# Autodesk Inventor assembly: POM_T5_15
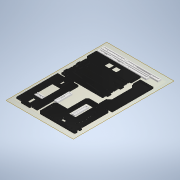
[picture p0: Inventor's stored thumbnail of the model, 180x180]
Saved by Autodesk Inventor 2020 (Build 240168000, 168)
## iProperties
Created: 2021-08-27
Part Number: POM_T5_15
Document SubType Name: Assembly
Designer: Masato
Author: Masato
## Documents named in this file (16)
- C:\Inventor\SUSTAINA-OP_0521\Cam\POM_T5_15.iam
- C:\Inventor\SUSTAINA-OP_0521\Cam\DisposableBoard.ipt
- C:\Inventor\SUSTAINA-OP_0521\UpperBody\Cockpit\Cockpit_battery_bottom_frame.ipt
- C:\Inventor\SUSTAINA-OP_0521\UpperBody\Cockpit\Cockpit_battery_front_frame.ipt
- C:\Inventor\SUSTAINA-OP_0521\UpperBody\Cockpit\Cockpit_side_frame.ipt
- C:\Inventor\SUSTAINA-OP_0521\UpperBody\Cockpit\Cockpit_back_frame.ipt
- C:\Inventor\SUSTAINA-OP_0521\UpperBody\Cockpit\Cockpit_battery_back_door.ipt
- C:\Inventor\SUSTAINA-OP_0521\UpperBody\Cockpit\Cockpit_top_frame.ipt
- C:\Inventor\SUSTAINA-OP_0521\Jig\Cockpit_side_frame_Jig.ipt
- C:\Inventor\SUSTAINA-OP_0521\Jig\Cockpit_battery_bottom_frame_Jig.ipt
- C:\Inventor\SUSTAINA-OP_0521\Jig\Cockpit_battery_back_door_Jig.ipt
- C:\Inventor\SUSTAINA-OP_0521\Jig\Cockpit_battery_front_frame_Jig.ipt
- C:\Inventor\SUSTAINA-OP_0521\Jig\Cockpit_battery_front_frame_Jig_2.ipt
- C:\Inventor\SUSTAINA-OP_0521\Jig\Cockpit_front_frame_Jig.ipt
- C:\Inventor\SUSTAINA-OP_0521\Jig\Cockpit_back_frame_Jig.ipt
- C:\Inventor\SUSTAINA-OP_0520\Jig\Cockpit_carrier_board_frame_Jig.ipt
## Components (15 placed, 15 different names)
1. DisposableBoard:1 — メイト:2, メイト:1, フラッシュ:1, フラッシュ:2, メイト:4, メイト:5, メイト:6, フラッシュ:3, フラッシュ:4, フラッシュ:6, メイト:7, メイト:8, メイト:12, メイト:14, メイト:17, メイト:20, メイト:26, メイト:27, メイト:28, メイト:32, メイト:33
2. Cockpit_side_frame:1 — メイト:5, フラッシュ:5, フラッシュ:6, フラッシュ:7, メイト:11, メイト:18, メイト:24, メイト:25
3. Cockpit_back_frame:1 — メイト:4, フラッシュ:3, フラッシュ:4, フラッシュ:5, フラッシュ:8, メイト:9, メイト:15, メイト:16, メイト:19
4. Cockpit_battery_back_door:1 — メイト:6, フラッシュ:7, メイト:11
5. Cockpit_battery_bottom_frame:1 — メイト:7, フラッシュ:8, フラッシュ:9, メイト:10, フラッシュ:10, メイト:13
6. Cockpit_battery_front_frame:1 — メイト:8, フラッシュ:9, メイト:9, メイト:10
7. Cockpit_top_frame:2 — メイト:12, フラッシュ:10, メイト:13, フラッシュ:13, メイト:29
8. Cockpit_side_frame_Jig:1 — メイト:14, メイト:15, メイト:16
9. Cockpit_battery_bottom_frame_Jig:1 — メイト:17, メイト:18, メイト:19
10. Cockpit_battery_back_door_Jig:1 — メイト:20, メイト:24, メイト:25
11. Cockpit_battery_front_frame_Jig:1 — メイト:26, フラッシュ:13, メイト:29, メイト:30, フラッシュ:14, フラッシュ:16, メイト:34
12. Cockpit_battery_front_frame_Jig_2:1 — メイト:27, メイト:30, フラッシュ:14, フラッシュ:15, メイト:31
13. Cockpit_front_frame_Jig:1 — メイト:28, フラッシュ:15, メイト:31
14. Cockpit_back_frame_Jig:1 — メイト:32, フラッシュ:16, メイト:34, フラッシュ:17, メイト:35
15. Cockpit_carrier_board_frame_Jig:1 — メイト:33, フラッシュ:17, メイト:35
## Relationships (46: Mate 31, Flush 15)
- メイト:2 [Mate]: DisposableBoard:1
- メイト:1 [Mate]: DisposableBoard:1
- フラッシュ:1 [Flush]: DisposableBoard:1
- フラッシュ:2 [Flush]: DisposableBoard:1
- メイト:4 [Mate]: DisposableBoard:1 ↔ Cockpit_back_frame:1
- メイト:5 [Mate]: DisposableBoard:1 ↔ Cockpit_side_frame:1
- メイト:6 [Mate]: DisposableBoard:1 ↔ Cockpit_battery_back_door:1
- フラッシュ:3 [Flush] (2 mm): DisposableBoard:1 ↔ Cockpit_back_frame:1
- フラッシュ:4 [Flush] (2 mm): DisposableBoard:1 ↔ Cockpit_back_frame:1
- フラッシュ:5 [Flush]: Cockpit_side_frame:1 ↔ Cockpit_back_frame:1
- フラッシュ:6 [Flush] (2 mm): DisposableBoard:1 ↔ Cockpit_side_frame:1
- フラッシュ:7 [Flush]: Cockpit_side_frame:1 ↔ Cockpit_battery_back_door:1
- メイト:7 [Mate]: DisposableBoard:1 ↔ Cockpit_battery_bottom_frame:1
- メイト:8 [Mate]: DisposableBoard:1 ↔ Cockpit_battery_front_frame:1
- フラッシュ:8 [Flush]: Cockpit_back_frame:1 ↔ Cockpit_battery_bottom_frame:1
- フラッシュ:9 [Flush]: Cockpit_battery_bottom_frame:1 ↔ Cockpit_battery_front_frame:1
- メイト:9 [Mate] (2.5 mm): Cockpit_back_frame:1 ↔ Cockpit_battery_front_frame:1
- メイト:10 [Mate] (2.5 mm): Cockpit_battery_bottom_frame:1 ↔ Cockpit_battery_front_frame:1
- メイト:11 [Mate] (2.5 mm): Cockpit_side_frame:1 ↔ Cockpit_battery_back_door:1
- メイト:12 [Mate]: DisposableBoard:1 ↔ Cockpit_top_frame:2
- フラッシュ:10 [Flush]: Cockpit_battery_bottom_frame:1 ↔ Cockpit_top_frame:2
- メイト:13 [Mate] (2.5 mm): Cockpit_battery_bottom_frame:1 ↔ Cockpit_top_frame:2
- メイト:14 [Mate]: DisposableBoard:1 ↔ Cockpit_side_frame_Jig:1
- メイト:15 [Mate] (2.5 mm): Cockpit_back_frame:1 ↔ Cockpit_side_frame_Jig:1
- メイト:16 [Mate] (3.5 mm): Cockpit_back_frame:1 ↔ Cockpit_side_frame_Jig:1
- メイト:17 [Mate]: DisposableBoard:1 ↔ Cockpit_battery_bottom_frame_Jig:1
- メイト:18 [Mate] (2.5 mm): Cockpit_side_frame:1 ↔ Cockpit_battery_bottom_frame_Jig:1
- メイト:19 [Mate] (2.5 mm): Cockpit_back_frame:1 ↔ Cockpit_battery_bottom_frame_Jig:1
- メイト:20 [Mate]: DisposableBoard:1 ↔ Cockpit_battery_back_door_Jig:1
- メイト:24 [Mate] (4.5 mm): Cockpit_side_frame:1 ↔ Cockpit_battery_back_door_Jig:1
- メイト:25 [Mate] (7 mm): Cockpit_side_frame:1 ↔ Cockpit_battery_back_door_Jig:1
- メイト:26 [Mate]: DisposableBoard:1 ↔ Cockpit_battery_front_frame_Jig:1
- メイト:27 [Mate]: DisposableBoard:1 ↔ Cockpit_battery_front_frame_Jig_2:1
- メイト:28 [Mate]: DisposableBoard:1 ↔ Cockpit_front_frame_Jig:1
- フラッシュ:13 [Flush]: Cockpit_top_frame:2 ↔ Cockpit_battery_front_frame_Jig:1
- メイト:29 [Mate] (2.5 mm): Cockpit_top_frame:2 ↔ Cockpit_battery_front_frame_Jig:1
- メイト:30 [Mate] (2.5 mm): Cockpit_battery_front_frame_Jig:1 ↔ Cockpit_battery_front_frame_Jig_2:1
- フラッシュ:14 [Flush]: Cockpit_battery_front_frame_Jig:1 ↔ Cockpit_battery_front_frame_Jig_2:1
- フラッシュ:15 [Flush]: Cockpit_battery_front_frame_Jig_2:1 ↔ Cockpit_front_frame_Jig:1
- メイト:31 [Mate] (2.5 mm): Cockpit_battery_front_frame_Jig_2:1 ↔ Cockpit_front_frame_Jig:1
- メイト:32 [Mate]: DisposableBoard:1 ↔ Cockpit_back_frame_Jig:1
- メイト:33 [Mate]: DisposableBoard:1 ↔ Cockpit_carrier_board_frame_Jig:1
- フラッシュ:16 [Flush]: Cockpit_battery_front_frame_Jig:1 ↔ Cockpit_back_frame_Jig:1
- メイト:34 [Mate] (2.5 mm): Cockpit_battery_front_frame_Jig:1 ↔ Cockpit_back_frame_Jig:1
- フラッシュ:17 [Flush]: Cockpit_back_frame_Jig:1 ↔ Cockpit_carrier_board_frame_Jig:1
- メイト:35 [Mate] (2.5 mm): Cockpit_back_frame_Jig:1 ↔ Cockpit_carrier_board_frame_Jig:1
